# Autodesk Inventor assembly: circulation pump
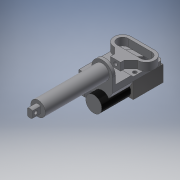
[picture p0: Inventor's stored thumbnail of the model, 180x180]
Saved by Autodesk Inventor 2017 (Build 210142000, 142)
## iProperties
Created: 2018-01-02
Part Number: circulation pump
Document SubType Name: Assembly
Designer: RLanting
Author: RLanting
## Documents named in this file (6)
- C:\Users\rmccomber\Documents\st motor\direct drive electronic valving 2\circulation pump\circulation pump.iam
- C:\Users\rmccomber\Documents\st motor\direct drive electronic valving 2\circulation pump\motor.ipt
- C:\Users\rmccomber\Documents\st motor\direct drive electronic valving 2\circulation pump\frame.ipt
- C:\Users\rmccomber\Documents\st motor\direct drive electronic valving 2\circulation pump\crank.ipt
- C:\Users\rmccomber\Documents\st motor\direct drive electronic valving 2\circulation pump\yoke.ipt
- C:\Users\rmccomber\Documents\st motor\direct drive electronic valving 2\circulation pump\cylinder.ipt
## Components (5 placed, 5 different names)
1. motor:1 — Mate:1, Mate:2, Mate:3, Mate:5
2. frame:1 — Mate:1, Mate:2, Mate:3, Mate:4, Mate:8, Mate:9
3. crank:1 — Mate:4, Mate:5, Tangent:1, Angle:2
4. yoke:1 — Tangent:1, Mate:10, Angle:1, Angle:2
5. cylinder:1 — Mate:8, Mate:9, Mate:10, Angle:1
## Relationships (11: Mate 8, Angle 2, Tangent 1)
- Mate:1: motor:1 ↔ frame:1
- Mate:2: motor:1 ↔ frame:1
- Mate:3: motor:1 ↔ frame:1
- Mate:4 (1 mm): frame:1 ↔ crank:1
- Mate:5: motor:1 ↔ crank:1
- Tangent:1 (7 mm): crank:1 ↔ yoke:1
- Mate:8: frame:1 ↔ cylinder:1
- Mate:9: frame:1 ↔ cylinder:1
- Mate:10: yoke:1 ↔ cylinder:1
- Angle:1 (180 deg): yoke:1 ↔ cylinder:1
- Angle:2 (0 deg): crank:1 ↔ yoke:1
